# Autodesk Inventor assembly: Assembly(A)
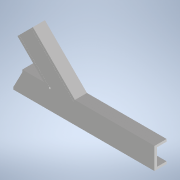
[picture p0: Inventor's stored thumbnail of the model, 180x180]
Saved by Autodesk Inventor 2020 (Build 240168000, 168)
## iProperties
Created: 2020-12-26
Part Number: Assembly(A)
Document SubType Name: Assembly
Designer: moham
Author: moham
## Documents named in this file (5)
- D:\Projects\MCT 131\The project\Track pieces\Section A\Assembly(A).iam
- D:\Projects\MCT 131\The project\Track pieces\Section A\A_Base.ipt
- D:\Projects\MCT 131\The project\Track pieces\Section A\A_LeftWall1(plan)_5.ipt
- D:\Projects\MCT 131\The project\Track pieces\Section A\A_LeftWall2(plan)_5.ipt
- D:\Projects\MCT 131\The project\Track pieces\Section A\A_RightWall.ipt
## Components (12 placed, 4 different names)
1. A_Base:1 — Mate:9, Mate:10, Flush:17, Flush:18, Mate:11, Mate:12, Mate:13, Flush:19, Flush:20
2. A_LeftWall1(plan)_5:1 — Flush:1, Flush:2, Mate:1, Flush:18, Mate:11, Mate:12
3. A_LeftWall1(plan)_5:2 — Flush:1, Flush:2, Flush:3, Flush:4, Mate:1, Mate:2
4. A_LeftWall1(plan)_5:3 — Flush:3, Flush:4, Flush:5, Flush:6, Mate:2, Mate:3
5. A_LeftWall1(plan)_5:4 — Flush:5, Flush:6, Flush:7, Flush:8, Mate:3, Mate:4
6. A_LeftWall1(plan)_5:5 — Flush:7, Flush:8, Mate:4
7. A_LeftWall2(plan)_5:1 — Flush:9, Flush:13, Mate:5, Mate:9, Mate:10, Flush:17
8. A_LeftWall2(plan)_5:2 — Flush:9, Flush:10, Flush:13, Flush:14, Mate:5, Mate:6
9. A_LeftWall2(plan)_5:3 — Flush:10, Flush:11, Flush:14, Flush:15, Mate:6, Mate:7
10. A_LeftWall2(plan)_5:4 — Flush:11, Flush:12, Flush:15, Flush:16, Mate:7, Mate:8
11. A_LeftWall2(plan)_5:5 — Flush:12, Flush:16, Mate:8
12. A_RightWall:1 — Mate:13, Flush:19, Flush:20
## Relationships (33: Flush 20, Mate 13)
- Flush:1: A_LeftWall1(plan)_5:1 ↔ A_LeftWall1(plan)_5:2
- Flush:2: A_LeftWall1(plan)_5:1 ↔ A_LeftWall1(plan)_5:2
- Flush:3: A_LeftWall1(plan)_5:2 ↔ A_LeftWall1(plan)_5:3
- Flush:4: A_LeftWall1(plan)_5:2 ↔ A_LeftWall1(plan)_5:3
- Flush:5: A_LeftWall1(plan)_5:3 ↔ A_LeftWall1(plan)_5:4
- Flush:6: A_LeftWall1(plan)_5:3 ↔ A_LeftWall1(plan)_5:4
- Flush:7: A_LeftWall1(plan)_5:4 ↔ A_LeftWall1(plan)_5:5
- Flush:8: A_LeftWall1(plan)_5:4 ↔ A_LeftWall1(plan)_5:5
- Mate:1: A_LeftWall1(plan)_5:1 ↔ A_LeftWall1(plan)_5:2
- Mate:2: A_LeftWall1(plan)_5:2 ↔ A_LeftWall1(plan)_5:3
- Mate:3: A_LeftWall1(plan)_5:3 ↔ A_LeftWall1(plan)_5:4
- Mate:4: A_LeftWall1(plan)_5:4 ↔ A_LeftWall1(plan)_5:5
- Flush:9: A_LeftWall2(plan)_5:1 ↔ A_LeftWall2(plan)_5:2
- Flush:10: A_LeftWall2(plan)_5:2 ↔ A_LeftWall2(plan)_5:3
- Flush:11: A_LeftWall2(plan)_5:3 ↔ A_LeftWall2(plan)_5:4
- Flush:12: A_LeftWall2(plan)_5:4 ↔ A_LeftWall2(plan)_5:5
- Flush:13: A_LeftWall2(plan)_5:1 ↔ A_LeftWall2(plan)_5:2
- Flush:14: A_LeftWall2(plan)_5:2 ↔ A_LeftWall2(plan)_5:3
- Flush:15: A_LeftWall2(plan)_5:3 ↔ A_LeftWall2(plan)_5:4
- Flush:16: A_LeftWall2(plan)_5:4 ↔ A_LeftWall2(plan)_5:5
- Mate:5: A_LeftWall2(plan)_5:1 ↔ A_LeftWall2(plan)_5:2
- Mate:6: A_LeftWall2(plan)_5:2 ↔ A_LeftWall2(plan)_5:3
- Mate:7: A_LeftWall2(plan)_5:3 ↔ A_LeftWall2(plan)_5:4
- Mate:8: A_LeftWall2(plan)_5:4 ↔ A_LeftWall2(plan)_5:5
- Mate:9: A_Base:1 ↔ A_LeftWall2(plan)_5:1
- Mate:10: A_Base:1 ↔ A_LeftWall2(plan)_5:1
- Flush:17: A_Base:1 ↔ A_LeftWall2(plan)_5:1
- Flush:18: A_Base:1 ↔ A_LeftWall1(plan)_5:1
- Mate:11: A_Base:1 ↔ A_LeftWall1(plan)_5:1
- Mate:12: A_Base:1 ↔ A_LeftWall1(plan)_5:1
- Mate:13: A_Base:1 ↔ A_RightWall:1
- Flush:19: A_Base:1 ↔ A_RightWall:1
- Flush:20: A_Base:1 ↔ A_RightWall:1
